# Autodesk Inventor assembly: LeftDriveTrainMecanum2017-18
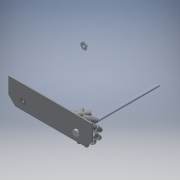
[picture p0: Inventor's stored thumbnail of the model, 180x180]
Saved by Autodesk Inventor 2017 (Build 210142000, 142)
## iProperties
Created: 2017-09-16
Part Number: LeftDriveTrainMecanum2017-18
Document SubType Name: Assembly
Designer: User
Author: User
## Documents named in this file (8)
- C:\Robotics\CAD\2016-17_CAD\Custom COTS\LeftDriveTrainMecanum2017-18.iam
- C:\Robotics\CAD\2017-18_CAD\MecanumDriveTrainPlate17-18.ipt
- C:\Robotics\CAD\COTSParts\Vex\HexBearings.5inchBore217-3875-STEP-20140818\HexBearings.5inchBore217-3875-STEP-20140818.ipt
- C:\Robotics\CAD\COTSParts\Vex\HexAxle.5inchOD217-3309-STEP\HexAxle.5inchOD18inchLength217-3309-STEP.ipt
- C:\Robotics\CAD\COTSParts\Vex\CollarClamp.5\am-1238+Collar+Clamp,+0.5''+Hex+Bore,+Aluminum.iam
- C:\Robotics\CAD\COTSParts\Vex\6inchMecanumLeft217-2799-STEP\6inchMecanumLeft217-2799.20121203.iam
- C:\Robotics\CAD\COTSParts\Vex\VersaHub.5inchBore217-4009-STEP-20140807\VersaHub.5inchBore217-4009-STEP-20140807.ipt
- C:\Robotics\CAD\COTSParts\Vex\HexSprocket.5inchBore\HexSprocket18t.5inchBore217-3488-STEP\HexSprocket18t.5inchBore217-3488-STEP.ipt
## Components (11 placed, 7 different names)
1. MecanumDriveTrainPlate17-18:1 — Mate:1, Mate:2, Mate:3, Mate:4, Mate:12
2. HexBearings.5inchBore217-3875-STEP-20140818:1 — Mate:1, Mate:2
3. HexBearings.5inchBore217-3875-STEP-20140818:2 — Mate:3, Mate:4, Mate:5, Mate:6, Mate:8
4. HexAxle.5inchOD18inchLength217-3309-STEP:1 — Mate:5, Mate:6, Mate:7, Mate:9, Flush:1, Mate:13, Mate:14, Mate:16, Mate:17
5. am-1238+Collar+Clamp,+0.5''+Hex+Bore,+Aluminum:1 [sub-assembly] — Mate:7, Mate:8, Mate:9, Flush:1
6. 6inchMecanumLeft217-2799.20121203:1 [sub-assembly] — Insert:1, Mate:10, Insert:2, Mate:11
7. VersaHub.5inchBore217-4009-STEP-20140807:1 — Insert:2, Mate:11, Mate:15
8. VersaHub.5inchBore217-4009-STEP-20140807:2 — Insert:1, Mate:10, Mate:16, Mate:17, Mate:18
9. am-1238+Collar+Clamp,+0.5''+Hex+Bore,+Aluminum:2 [sub-assembly] — Mate:18
10. am-1238+Collar+Clamp,+0.5''+Hex+Bore,+Aluminum:3 [sub-assembly] — Mate:12, Mate:13, Mate:14, Mate:15
11. HexSprocket18t.5inchBore217-3488-STEP:1
## Relationships (21: Mate 18, Insert 2, Flush 1)
- Mate:1: MecanumDriveTrainPlate17-18:1 ↔ HexBearings.5inchBore217-3875-STEP-20140818:1
- Mate:2: MecanumDriveTrainPlate17-18:1 ↔ HexBearings.5inchBore217-3875-STEP-20140818:1
- Mate:3: MecanumDriveTrainPlate17-18:1 ↔ HexBearings.5inchBore217-3875-STEP-20140818:2
- Mate:4: MecanumDriveTrainPlate17-18:1 ↔ HexBearings.5inchBore217-3875-STEP-20140818:2
- Mate:5: HexBearings.5inchBore217-3875-STEP-20140818:2 ↔ HexAxle.5inchOD18inchLength217-3309-STEP:1
- Mate:6: HexBearings.5inchBore217-3875-STEP-20140818:2 ↔ HexAxle.5inchOD18inchLength217-3309-STEP:1
- Mate:7: HexAxle.5inchOD18inchLength217-3309-STEP:1 ↔ am-1238+Collar+Clamp,+0.5''+Hex+Bore,+Aluminum:1
- Mate:8: HexBearings.5inchBore217-3875-STEP-20140818:2 ↔ am-1238+Collar+Clamp,+0.5''+Hex+Bore,+Aluminum:1
- Mate:9: HexAxle.5inchOD18inchLength217-3309-STEP:1 ↔ am-1238+Collar+Clamp,+0.5''+Hex+Bore,+Aluminum:1
- Flush:1: HexAxle.5inchOD18inchLength217-3309-STEP:1 ↔ am-1238+Collar+Clamp,+0.5''+Hex+Bore,+Aluminum:1
- Insert:1: 6inchMecanumLeft217-2799.20121203:1 ↔ VersaHub.5inchBore217-4009-STEP-20140807:2
- Mate:10: 6inchMecanumLeft217-2799.20121203:1 ↔ VersaHub.5inchBore217-4009-STEP-20140807:2
- Insert:2: 6inchMecanumLeft217-2799.20121203:1 ↔ VersaHub.5inchBore217-4009-STEP-20140807:1
- Mate:11: 6inchMecanumLeft217-2799.20121203:1 ↔ VersaHub.5inchBore217-4009-STEP-20140807:1
- Mate:12 (3.175 mm): MecanumDriveTrainPlate17-18:1 ↔ am-1238+Collar+Clamp,+0.5''+Hex+Bore,+Aluminum:3
- Mate:13: HexAxle.5inchOD18inchLength217-3309-STEP:1 ↔ am-1238+Collar+Clamp,+0.5''+Hex+Bore,+Aluminum:3
- Mate:14: HexAxle.5inchOD18inchLength217-3309-STEP:1 ↔ am-1238+Collar+Clamp,+0.5''+Hex+Bore,+Aluminum:3
- Mate:15: VersaHub.5inchBore217-4009-STEP-20140807:1 ↔ am-1238+Collar+Clamp,+0.5''+Hex+Bore,+Aluminum:3
- Mate:16: HexAxle.5inchOD18inchLength217-3309-STEP:1 ↔ VersaHub.5inchBore217-4009-STEP-20140807:2
- Mate:17: HexAxle.5inchOD18inchLength217-3309-STEP:1 ↔ VersaHub.5inchBore217-4009-STEP-20140807:2
- Mate:18: VersaHub.5inchBore217-4009-STEP-20140807:2 ↔ am-1238+Collar+Clamp,+0.5''+Hex+Bore,+Aluminum:2
